# Autodesk Inventor assembly: Valve2.5
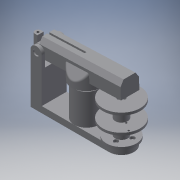
[picture p0: Inventor's stored thumbnail of the model, 180x180]
Saved by Autodesk Inventor 2019 (Build 230136000, 136)
## iProperties
Created: 2019-02-21
Part Number: Valve2.5
Document SubType Name: Assembly
Designer: Kepler
Author: Kepler
## Documents named in this file (5)
- C:\Users\Kepler\Documents\Inventor\Organ Valves\OrganValveMk2\Valve2.5.iam
- C:\Users\Kepler\Documents\Inventor\Organ Valves\OrganValveMk2\Axel Mk2.ipt
- C:\Users\Kepler\Documents\Inventor\Organ Valves\OrganValveMk2\SpoolMk2.ipt
- C:\Users\Kepler\Documents\Inventor\Organ Valves\OrganValveMk2\ValveHeadMk2.5.ipt
- C:\Users\Kepler\Documents\Inventor\Organ Valves\OrganValveMk2\ValveBaseMk2.5.ipt
## Components (4 placed, 4 different names)
1. Axel Mk2:1 — Mate:5, Mate:6
2. SpoolMk2:1 — Mate:7, Mate:8
3. ValveHeadMk2.5:1 — Mate:5, Mate:9
4. ValveBaseMk2.5:1 — Mate:6, Mate:7, Mate:8, Mate:9
## Relationships (5: Mate 5)
- Mate:5: Axel Mk2:1 ↔ ValveHeadMk2.5:1
- Mate:6: Axel Mk2:1 ↔ ValveBaseMk2.5:1
- Mate:7: SpoolMk2:1 ↔ ValveBaseMk2.5:1
- Mate:8: SpoolMk2:1 ↔ ValveBaseMk2.5:1
- Mate:9 (0.15 mm): ValveHeadMk2.5:1 ↔ ValveBaseMk2.5:1
